# Autodesk Inventor assembly: Full Carousel Assembly
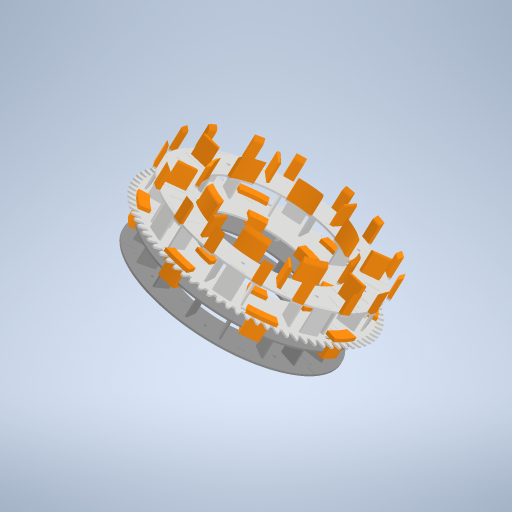
[picture p0: Inventor's stored thumbnail of the model, 512x512]
Saved by Autodesk Inventor 2023 (Build 270158000, 158)
## iProperties
Created: 2023-02-14
Part Number: Full Carousel Assembly
Document SubType Name: Assembly
Designer: cheng
Author: cheng
## Documents named in this file (3)
- C:\Users\mihal\Desktop\4th Year Project\Final Assembly\Complete Carousel Assembly.iam
- C:\Users\mihal\Desktop\4th Year Project\Final Assembly\Rotating Carousel\Moving Carousel Assembly.iam
- C:\Users\mihal\Desktop\4th Year Project\Final Assembly\Non-Rotating Carousel\Non-Rotating Carousel Assembly.iam
## Components (2 placed, 2 different names)
1. Non-Rotating Carousel Assembly:1 [sub-assembly] — Mate:1, Mate:2
2. Moving Carousel Assembly:2 [sub-assembly] — Mate:1, Mate:2
## Relationships (2: Mate 2)
- Mate:1: Non-Rotating Carousel Assembly:1 ↔ Moving Carousel Assembly:2
- Mate:2: Non-Rotating Carousel Assembly:1 ↔ Moving Carousel Assembly:2
